# Autodesk Inventor assembly: allvany2
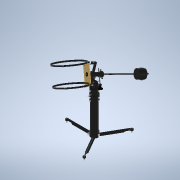
[picture p0: Inventor's stored thumbnail of the model, 180x180]
Saved by Autodesk Inventor 2021.4 (Build 254397000, 397)
## iProperties
Created: 2023-11-18
Part Number: allvany2
Document SubType Name: Assembly
Designer: vtoth
Author: vtoth
## Documents named in this file (17)
- C:\Users\vtoth\OneDrive - Budapesti Műszaki és Gazdaságtudományi Egyetem\5_felev\CAD\hf2_v2\allvany2.iam
- C:\Users\vtoth\OneDrive - Budapesti Műszaki és Gazdaságtudományi Egyetem\5_felev\CAD\hf2_v2\skeleton_1.ipt
- C:\Users\vtoth\OneDrive - Budapesti Műszaki és Gazdaságtudományi Egyetem\5_felev\CAD\hf2_v2\DEC_tengely.ipt
- C:\Users\vtoth\OneDrive - Budapesti Műszaki és Gazdaságtudományi Egyetem\5_felev\CAD\hf2_v2\forgoresz.iam
- C:\Users\vtoth\OneDrive - Budapesti Műszaki és Gazdaságtudományi Egyetem\5_felev\CAD\hf2_v2\polus.iam
- C:\Users\vtoth\OneDrive - Budapesti Műszaki és Gazdaságtudományi Egyetem\5_felev\CAD\hf2_v2\RA_haz.iam
- C:\Users\vtoth\OneDrive - Budapesti Műszaki és Gazdaságtudományi Egyetem\5_felev\CAD\hf2_v2\DEC_haz.iam
- C:\Users\vtoth\OneDrive - Budapesti Műszaki és Gazdaságtudományi Egyetem\5_felev\CAD\hf2_v2\RA_csavar.ipt
- C:\Users\vtoth\OneDrive - Budapesti Műszaki és Gazdaságtudományi Egyetem\5_felev\CAD\hf2_v2\tavcsofogo.iam
- C:\Users\vtoth\OneDrive - Budapesti Műszaki és Gazdaságtudományi Egyetem\5_felev\CAD\hf2_v2\DEC_csavar.ipt
- C:\Users\vtoth\OneDrive - Budapesti Műszaki és Gazdaságtudományi Egyetem\5_felev\CAD\hf2_v2\knob.ipt
- C:\Users\vtoth\OneDrive - Budapesti Műszaki és Gazdaságtudományi Egyetem\5_felev\CAD\hf2_v2\talp.iam
- C:\Users\vtoth\OneDrive - Budapesti Műszaki és Gazdaságtudományi Egyetem\5_felev\CAD\hf2_v2\ellensuly.iam
- C:\Users\vtoth\OneDrive - Budapesti Műszaki és Gazdaságtudományi Egyetem\5_felev\CAD\hf2_v2\ContentCenter\en-US\ISO 4018\ISO 4018 - M12 x 70.ipt
- C:\Users\vtoth\OneDrive - Budapesti Műszaki és Gazdaságtudományi Egyetem\5_felev\CAD\hf2_v2\ContentCenter\en-US\ISO 4032(2)\ISO 4032 - M12 - ISO.ipt
- C:\Users\vtoth\OneDrive - Budapesti Műszaki és Gazdaságtudományi Egyetem\5_felev\CAD\hf2_v2\ContentCenter\en-US\DIN EN ISO 7091\DIN EN ISO 7091 - 12.ipt
- C:\Users\vtoth\OneDrive - Budapesti Műszaki és Gazdaságtudományi Egyetem\5_felev\CAD\hf2_v2\skeleton_2.ipt
## Components (17 placed, 15 different names)
1. talp:2 [sub-assembly] — Mate:4, Mate:5, Flush:3, Insert:1, Tangent:1
2. forgoresz:2 [sub-assembly] — Insert:1, Insert:2, Tangent:1, Mate:1, Tangent:2
3. polus:2 [sub-assembly] — Insert:2, Insert:3, Mate:1, Tangent:2, Insert:12
4. RA_haz:2 [sub-assembly] — Insert:3, Angle:1, Insert:6, Insert:9, Insert:13, Insert:19, Mate:9
5. DEC_haz:2 [sub-assembly] — Angle:2, Insert:5, Insert:19, Mate:6, Mate:7, Mate:8, Mate:11
6. DEC_tengely:1 — Insert:5, Insert:18, Insert:22
7. tavcsofogo:1 [sub-assembly] — Insert:20, Insert:21, Insert:22, Mate:10
8. ellensuly:1 [sub-assembly] — Insert:18
9. RA_csavar:1 — Insert:6, Mate:6, Mate:12
10. DEC_csavar:1 — Insert:20, Mate:7
11. knob:1 — Insert:21
12. knob:2 — Insert:9
13. ISO 4018 M12 x 70:1
14. ISO 4032 M12:1 — Insert:12
15. ISO 4032 M12:2 — Insert:14
16. DIN EN ISO 7091 12:1 — Insert:13, Insert:14
17. skeleton_2:1 — Flush:4, Flush:5, Flush:6, Angle:1, Angle:2, Mate:8, Mate:9, Mate:10, Mate:11, Mate:12
## Relationships (34: Insert 15, Mate 10, Flush 4, Angle 3, Tangent 2)
- Mate:4: talp:2
- Mate:5: talp:2
- Flush:3: talp:2
- Insert:1: talp:2 ↔ forgoresz:2
- Flush:4: skeleton_2:1
- Flush:5: skeleton_2:1
- Flush:6: skeleton_2:1
- Insert:2: forgoresz:2 ↔ polus:2
- Insert:3: polus:2 ↔ RA_haz:2
- Angle:1 (0 deg): RA_haz:2 ↔ skeleton_2:1
- Angle:2 (180 deg): DEC_haz:2 ↔ skeleton_2:1
- Insert:5: DEC_haz:2 ↔ DEC_tengely:1
- Tangent:1: talp:2 ↔ forgoresz:2
- Mate:1: forgoresz:2 ↔ polus:2
- Tangent:2: forgoresz:2 ↔ polus:2
- Insert:6: RA_haz:2 ↔ RA_csavar:1
- Insert:9: RA_haz:2 ↔ knob:2
- [Insert]: polus:2 ↔ ISO 4018 M12 x 70:1
- Insert:12: polus:2 ↔ ISO 4032 M12:1
- [Angle] (0 deg): ISO 4018 M12 x 70:1 ↔ ISO 4032 M12:1
- Insert:13: RA_haz:2 ↔ DIN EN ISO 7091 12:1
- Insert:14: ISO 4032 M12:2 ↔ DIN EN ISO 7091 12:1
- Insert:18: DEC_tengely:1 ↔ ellensuly:1
- Insert:19: RA_haz:2 ↔ DEC_haz:2
- Mate:6: DEC_haz:2 ↔ RA_csavar:1
- Insert:20: tavcsofogo:1 ↔ DEC_csavar:1
- Insert:21: tavcsofogo:1 ↔ knob:1
- Mate:7: DEC_haz:2 ↔ DEC_csavar:1
- Insert:22: DEC_tengely:1 ↔ tavcsofogo:1
- Mate:8: DEC_haz:2 ↔ skeleton_2:1
- Mate:9: RA_haz:2 ↔ skeleton_2:1
- Mate:10: tavcsofogo:1 ↔ skeleton_2:1
- Mate:11: DEC_haz:2 ↔ skeleton_2:1
- Mate:12: RA_csavar:1 ↔ skeleton_2:1
## Named parameters: polus = 47 deg, DEC = 0 deg, RA = 0 deg
